# Autodesk Inventor assembly: Tool Holder Assembly
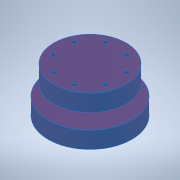
[picture p0: Inventor's stored thumbnail of the model, 180x180]
Saved by Autodesk Inventor 2022 (Build 260153000, 153)
## iProperties
Created: 2021-04-16
Part Number: Tool Holder Assembly
Document SubType Name: Assembly
Designer: caleb
Author: caleb
## Documents named in this file (4)
- C:\Users\Caleb\Desktop\nebraska-silicon-lab\Hardware\General Gantry\Gantry Tool Holder - Phase II\Tool Holder Assembly.iam
- C:\Users\Caleb\Desktop\nebraska-silicon-lab\Hardware\General Gantry\Gantry Tool Holder - Phase II\ToolHolder1.ipt
- C:\Users\Caleb\Desktop\nebraska-silicon-lab\Hardware\General Gantry\Gantry Tool Holder - Phase II\9396K153 Silicone O-Ring .ipt
- C:\Users\Caleb\Desktop\nebraska-silicon-lab\Hardware\General Gantry\Gantry Tool Holder - Phase II\9396K27 Silicone O-Ring.ipt
## Components (3 placed, 3 different names)
1. ToolHolder1:1 — Insert:1
2. 9396K153 Silicone O-Ring :1 — Insert:1
3. 9396K27 Silicone O-Ring:1
## Relationships (1: Insert 1)
- Insert:1: ToolHolder1:1 ↔ 9396K153 Silicone O-Ring :1
